# Autodesk Inventor assembly: Samlet_Projekt
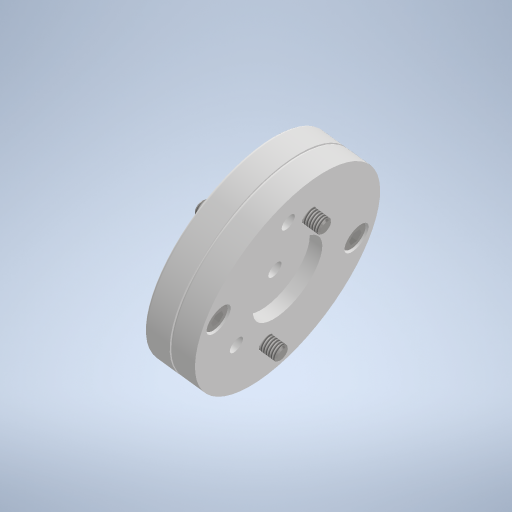
[picture p0: Inventor's stored thumbnail of the model, 512x512]
Saved by Autodesk Inventor 2024 (Build 280153000, 153)
## iProperties
Created: 2024-03-07
Part Number: Samlet_Projekt
Document SubType Name: Assembly
Designer: jona3
Author: jona3
## Documents named in this file (5)
- C:\Users\jona3\OneDrive\Dokumenter\Inventor\Første dims\Samlet_Projekt.iam
- C:\Users\jona3\OneDrive\Dokumenter\Inventor\Første dims\Part1-frfr.ipt
- C:\Users\jona3\OneDrive\Dokumenter\Inventor\Første dims\Part2_small.ipt
- C:\Users\jona3\OneDrive\Dokumenter\Inventor\Content Center Files\R2024\en-US\DIN 912\DIN 912 - M6 x 1 x 10 x 7,5.ipt
- C:\Users\jona3\OneDrive\Dokumenter\Inventor\Content Center Files\R2024\en-US\DIN 912\DIN 912 - M6 x 1 x 12 x 9,5.ipt
## Components (10 placed, 4 different names)
1. Part1-frfr:1 — Insert:1, Insert:2, Insert:3, Insert:4, Mate:1, Mate:2, Mate:3
2. Part2_small:1 — Insert:5, Insert:6, Mate:1, Mate:2, Mate:3, Insert:7, Insert:8
3. DIN 912 - replaced by DIN EN ISO 4762 M6 x 10:1 — Insert:1
4. DIN 912 - replaced by DIN EN ISO 4762 M6 x 10:2 — Insert:2
5. DIN 912 - replaced by DIN EN ISO 4762 M6 x 10:3 — Insert:3
6. DIN 912 - replaced by DIN EN ISO 4762 M6 x 10:4 — Insert:4
7. DIN 912 - replaced by DIN EN ISO 4762 M6 x 10:5 — Insert:5
8. DIN 912 - replaced by DIN EN ISO 4762 M6 x 10:6 — Insert:6
9. DIN 912 - replaced by DIN EN ISO 4762 M6 x 12:1 — Insert:7
10. DIN 912 - replaced by DIN EN ISO 4762 M6 x 10:8 — Insert:8
## Relationships (11: Insert 8, Mate 3)
- Insert:1: Part1-frfr:1 ↔ DIN 912 - replaced by DIN EN ISO 4762 M6 x 10:1
- Insert:2: Part1-frfr:1 ↔ DIN 912 - replaced by DIN EN ISO 4762 M6 x 10:2
- Insert:3: Part1-frfr:1 ↔ DIN 912 - replaced by DIN EN ISO 4762 M6 x 10:3
- Insert:4: Part1-frfr:1 ↔ DIN 912 - replaced by DIN EN ISO 4762 M6 x 10:4
- Insert:5: Part2_small:1 ↔ DIN 912 - replaced by DIN EN ISO 4762 M6 x 10:5
- Insert:6: Part2_small:1 ↔ DIN 912 - replaced by DIN EN ISO 4762 M6 x 10:6
- Mate:1: Part1-frfr:1 ↔ Part2_small:1
- Mate:2: Part1-frfr:1 ↔ Part2_small:1
- Mate:3: Part1-frfr:1 ↔ Part2_small:1
- Insert:7: Part2_small:1 ↔ DIN 912 - replaced by DIN EN ISO 4762 M6 x 12:1
- Insert:8: Part2_small:1 ↔ DIN 912 - replaced by DIN EN ISO 4762 M6 x 10:8
